# Autodesk Inventor assembly: CW_ASSY
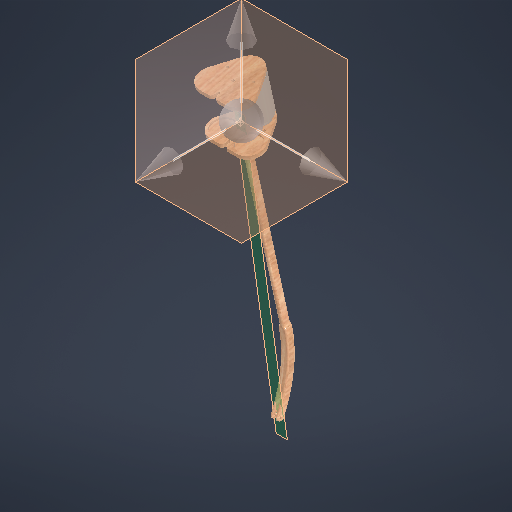
[picture p0: Inventor's stored thumbnail of the model, 512x512]
Saved by Autodesk Inventor 2026.2 (Build 302298010, 298A)
## iProperties
Created: 2026-02-25
Part Number: CW_ASSY
Document SubType Name: Assembly
Designer: 4aida
Mass: 1016.17 g
Surface Area: 2684.18 cm^2
Volume: 613.87 cm^3
Density: 1.65534 g/cm^3
Author: 4aida
## Documents named in this file (7)
- C:\Users\4aida\OneDrive\Documents\GitHub\Design_II_Group6\Trebuchet\WIPPER_TREBUCHET\CW_ASSY.iam
- C:\Users\4aida\OneDrive\Documents\GitHub\Design_II_Group6\Trebuchet\COUNTERWEIGHT_OUTSIDE_ARM,TREBUCHET.ipt
- C:\Users\4aida\OneDrive\Documents\GitHub\Design_II_Group6\Trebuchet\WIPPER_TREBUCHET\BOTTOM_PLATE_WEIGHTS_TREBUCHET.ipt
- C:\Users\4aida\OneDrive\Documents\GitHub\Design_II_Group6\Trebuchet\WIPPER_TREBUCHET\CW_PIVOT_TREBUCHET.ipt
- C:\Users\4aida\OneDrive\Documents\GitHub\Design_II_Group6\Trebuchet\WIPPER_TREBUCHET\TOP_PLATE_WEIGHTS_TREBUCHET.ipt
- C:\Users\4aida\OneDrive\Documents\GitHub\Design_II_Group6\Trebuchet\Canette-355ml.ipt
- C:\Users\4aida\OneDrive\Documents\GitHub\Design_II_Group6\Trebuchet\WIPPER_TREBUCHET\CONTERWEIGHT_SHAFT_TREBUCHET.ipt
## Components (8 placed, 6 different names)
1. COUNTERWEIGHT_OUTSIDE_ARM,TREBUCHET:1 — Mate:10
2. BOTTOM_PLATE_WEIGHTS_TREBUCHET:1
3. CW_PIVOT_TREBUCHET:1 — Tangent:1
4. TOP_PLATE_WEIGHTS_TREBUCHET:1
5. Canette-355ml:1
6. Canette-355ml:2
7. Canette-355ml:3
8. CONTERWEIGHT_SHAFT_TREBUCHET:1
## Relationships (16: Mate 10, Flush 4, Insert 1, Tangent 1)
- [Mate]: COUNTERWEIGHT_OUTSIDE_ARM,TREBUCHET:1 ↔ CW_PIVOT_TREBUCHET:1
- [Mate]: COUNTERWEIGHT_OUTSIDE_ARM,TREBUCHET:1 ↔ TOP_PLATE_WEIGHTS_TREBUCHET:1
- [Mate]: COUNTERWEIGHT_OUTSIDE_ARM,TREBUCHET:1 ↔ TOP_PLATE_WEIGHTS_TREBUCHET:1
- [Mate]: COUNTERWEIGHT_OUTSIDE_ARM,TREBUCHET:1 ↔ TOP_PLATE_WEIGHTS_TREBUCHET:1
- [Mate]: TOP_PLATE_WEIGHTS_TREBUCHET:1 ↔ Canette-355ml:1
- [Mate]: TOP_PLATE_WEIGHTS_TREBUCHET:1 ↔ Canette-355ml:3
- [Mate]: TOP_PLATE_WEIGHTS_TREBUCHET:1 ↔ Canette-355ml:2
- [Flush]: Canette-355ml:1 ↔ Canette-355ml:2
- [Flush]: Canette-355ml:1 ↔ Canette-355ml:3
- [Mate]: TOP_PLATE_WEIGHTS_TREBUCHET:1 ↔ Canette-355ml:1
- [Flush]: BOTTOM_PLATE_WEIGHTS_TREBUCHET:1 ↔ TOP_PLATE_WEIGHTS_TREBUCHET:1
- [Flush]: BOTTOM_PLATE_WEIGHTS_TREBUCHET:1 ↔ TOP_PLATE_WEIGHTS_TREBUCHET:1
- [Mate] (112 mm): BOTTOM_PLATE_WEIGHTS_TREBUCHET:1 ↔ TOP_PLATE_WEIGHTS_TREBUCHET:1
- [Insert]: COUNTERWEIGHT_OUTSIDE_ARM,TREBUCHET:1 ↔ CONTERWEIGHT_SHAFT_TREBUCHET:1
- Mate:10: COUNTERWEIGHT_OUTSIDE_ARM,TREBUCHET:1
- Tangent:1: CW_PIVOT_TREBUCHET:1
